# Autodesk Inventor assembly: handAssembly
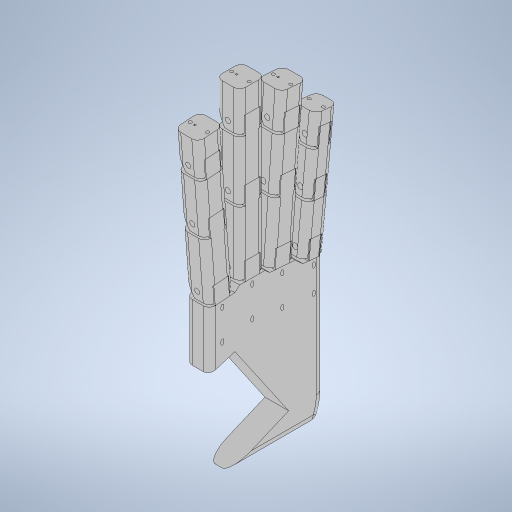
[picture p0: Inventor's stored thumbnail of the model, 512x512]
Saved by Autodesk Inventor 2024 (Build 280153000, 153)
## iProperties
Created: 2024-06-09
Part Number: handAssembly
Document SubType Name: Assembly
Designer: omiye
Author: omiye
## Documents named in this file (13)
- C:\Projects\roboticHand\fingerModels\handAssembly.iam
- C:\Projects\roboticHand\fingerModels\palm.ipt
- C:\Projects\roboticHand\fingerModels\normMale.ipt
- C:\Projects\roboticHand\fingerModels\fingerIndexRing\lower.ipt
- C:\Projects\roboticHand\fingerModels\fingerIndexRing\middle.ipt
- C:\Projects\roboticHand\fingerModels\fingerIndexRing\top.ipt
- C:\Projects\roboticHand\fingerModels\fingerMiddle\middle.ipt
- C:\Projects\roboticHand\fingerModels\fingerMiddle\top.ipt
- C:\Projects\roboticHand\fingerModels\fingerMiddle\lower.ipt
- C:\Projects\roboticHand\fingerModels\pinkyMale.ipt
- C:\Projects\roboticHand\fingerModels\fingerPinky\lower.ipt
- C:\Projects\roboticHand\fingerModels\fingerPinky\middle.ipt
- C:\Projects\roboticHand\fingerModels\fingerPinky\top.ipt
## Components (17 placed, 6 different names)
1. palm:1 — Mate:1, Mate:2, Mate:3, Mate:4, Mate:5, Mate:6, Mate:7, Mate:8, Mate:9, Mate:10, Mate:11, Mate:42, Mate:43, Mate:44
2. normMale:1 — Mate:1, Mate:2, Mate:3, Mate:4, Mate:5, Mate:33, Mate:34, Mate:35
3. normMale:2 — Mate:9, Mate:10, Mate:11, Mate:21, Mate:22, Mate:23
4. normMale:4 — Mate:6, Mate:7, Mate:8, Mate:24, Mate:25, Mate:26
5. lower:1 — Mate:15, Mate:16, Mate:17, Mate:21, Mate:22, Mate:23
6. middle:1 — Mate:15, Mate:16, Mate:17, Mate:18, Mate:19, Mate:20
7. top:1 — Mate:18, Mate:19, Mate:20
8. middle:2 — Mate:27, Mate:28, Mate:29, Mate:30, Mate:31, Mate:32
9. top:2 — Mate:30, Mate:31, Mate:32
10. lower:2 — Mate:24, Mate:25, Mate:26, Mate:27, Mate:28, Mate:29
11. middle:3 — Mate:36, Mate:37, Mate:38, Mate:39, Mate:40, Mate:41
12. top:3 — Mate:39, Mate:40, Mate:41
13. lower:3 — Mate:33, Mate:34, Mate:35, Mate:36, Mate:37, Mate:38
14. pinkyMale:1 — Mate:42, Mate:43, Mate:44, Mate:45, Mate:46, Mate:47
15. lower:4 — Mate:45, Mate:46, Mate:47, Mate:48, Mate:49, Mate:50
16. middle:4 — Mate:48, Mate:49, Mate:50, Mate:51, Mate:52, Mate:53
17. top:4 — Mate:51, Mate:52, Mate:53
## Relationships (50: Mate 50)
- Mate:1: palm:1 ↔ normMale:1
- Mate:2: palm:1 ↔ normMale:1
- Mate:3: palm:1 ↔ normMale:1
- Mate:4: palm:1 ↔ normMale:1
- Mate:5: palm:1 ↔ normMale:1
- Mate:6: palm:1 ↔ normMale:4
- Mate:7: palm:1 ↔ normMale:4
- Mate:8: palm:1 ↔ normMale:4
- Mate:9: palm:1 ↔ normMale:2
- Mate:10: palm:1 ↔ normMale:2
- Mate:11: palm:1 ↔ normMale:2
- Mate:15: lower:1 ↔ middle:1
- Mate:16: lower:1 ↔ middle:1
- Mate:17: lower:1 ↔ middle:1
- Mate:18: middle:1 ↔ top:1
- Mate:19: middle:1 ↔ top:1
- Mate:20: middle:1 ↔ top:1
- Mate:21: normMale:2 ↔ lower:1
- Mate:22: normMale:2 ↔ lower:1
- Mate:23: normMale:2 ↔ lower:1
- Mate:24: normMale:4 ↔ lower:2
- Mate:25: normMale:4 ↔ lower:2
- Mate:26: normMale:4 ↔ lower:2
- Mate:27: middle:2 ↔ lower:2
- Mate:28: middle:2 ↔ lower:2
- Mate:29: middle:2 ↔ lower:2
- Mate:30: middle:2 ↔ top:2
- Mate:31: middle:2 ↔ top:2
- Mate:32: middle:2 ↔ top:2
- Mate:33: normMale:1 ↔ lower:3
- Mate:34: normMale:1 ↔ lower:3
- Mate:35: normMale:1 ↔ lower:3
- Mate:36: middle:3 ↔ lower:3
- Mate:37: middle:3 ↔ lower:3
- Mate:38: middle:3 ↔ lower:3
- Mate:39: middle:3 ↔ top:3
- Mate:40: middle:3 ↔ top:3
- Mate:41: middle:3 ↔ top:3
- Mate:42: palm:1 ↔ pinkyMale:1
- Mate:43: palm:1 ↔ pinkyMale:1
- Mate:44: palm:1 ↔ pinkyMale:1
- Mate:45: pinkyMale:1 ↔ lower:4
- Mate:46: pinkyMale:1 ↔ lower:4
- Mate:47: pinkyMale:1 ↔ lower:4
- Mate:48: lower:4 ↔ middle:4
- Mate:49: lower:4 ↔ middle:4
- Mate:50: lower:4 ↔ middle:4
- Mate:51: middle:4 ↔ top:4
- Mate:52: middle:4 ↔ top:4
- Mate:53: middle:4 ↔ top:4
